# Autodesk Inventor assembly: collector wheel mounted on low channel
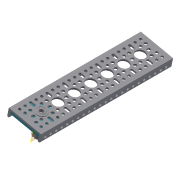
[picture p0: Inventor's stored thumbnail of the model, 180x180]
Saved by Autodesk Inventor 2018 (Build 220112000, 112)
## iProperties
Created: 2019-02-06
Part Number: collector wheel mounted on low channel
Document SubType Name: Assembly
Designer: ball
Author: ball
## Documents named in this file (6)
- C:\FTC\FTC8863CAD\2018Robot\collector wheel mounted on low channel.iam
- C:\FTC\FTC8863CAD\GoBilda\1121 Parts\1121-0007-0192.ipt
- C:\FTC\FTC8863CAD\2018Robot\Floor.ipt
- C:\FTC\FTC8863CAD\GoBilda\1601 Parts\1601-0014-0006.ipt
- C:\FTC\FTC8863CAD\2018Robot\CasterBallTemp.ipt
- C:\FTC\FTC8863CAD\2018Robot\BallMount.ipt
## Components (5 placed, 5 different names)
1. 1121-0007-0192:1 — Mate:1, Flush:1, Angle:1, Mate:6, Mate:7, Flush:2
2. Floor:1 — Mate:1, Flush:1, Angle:1
3. 1601-0014-0006:1 — Mate:6, Mate:7
4. CasterBallTemp:2 — Mate:8
5. BallMount:1 — Flush:2, Mate:8
## Relationships (7: Mate 4, Flush 2, Angle 1)
- Mate:1 (4.572 mm): 1121-0007-0192:1 ↔ Floor:1
- Flush:1: 1121-0007-0192:1 ↔ Floor:1
- Angle:1 (166 deg): 1121-0007-0192:1 ↔ Floor:1
- Mate:6: 1121-0007-0192:1 ↔ 1601-0014-0006:1
- Mate:7: 1121-0007-0192:1 ↔ 1601-0014-0006:1
- Flush:2: 1121-0007-0192:1 ↔ BallMount:1
- Mate:8: CasterBallTemp:2 ↔ BallMount:1
